# Autodesk Inventor assembly: Sun_StarwarsTrain
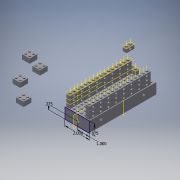
[picture p0: Inventor's stored thumbnail of the model, 180x180]
Saved by Autodesk Inventor 2016 (Build 200138000, 138)
## iProperties
Created: 2018-02-15
Part Number: Sun_StarwarsTrain
Document SubType Name: Assembly
Designer: sun01147
Author: sun01147
## Documents named in this file (6)
- E:\IED7_SunT\BrickTrainParts\Sun_StarwarsTrain.iam
- E:\IED7_SunT\BrickTrainParts\Caufield_Engine_Body_LEGO.ipt
- E:\IED7_SunT\BrickTrainParts\Sun_Bricks.ipt
- E:\IED7_SunT\BrickTrainParts\Yee_2x2Brick.ipt
- E:\IED7_SunT\BrickTrainParts\Sun_Bricks_MIR.ipt
- E:\IED7_SunT\BrickTrainParts\Sun_Bricks_MIR1.ipt
## Components (56 placed, 5 different names)
1. Caufield_Engine_Body_LEGO:1 — Mate:7, Mate:8, Mate:55
2. Sun_Bricks:1 — Mate:9, Flush:1, Mate:10, Flush:2, Flush:11
3. Sun_Bricks:2 — Mate:7, Mate:8, Mate:9, Flush:1, Mate:16
4. Sun_Bricks:3 — Mate:10, Flush:2, Flush:3, Mate:11, Mate:19
5. Sun_Bricks:4 — Flush:3, Mate:11, Mate:12, Flush:4, Mate:36
6. Yee_2x2Brick:1
7. Yee_2x2Brick:2
8. Yee_2x2Brick:3
9. Yee_2x2Brick:4
10. Sun_Bricks:5 — Mate:13, Flush:5, Mate:14, Flush:6
11. Sun_Bricks:6 — Mate:12, Flush:4, Mate:13, Flush:5
12. Sun_Bricks:7 — Mate:14, Flush:6, Mate:15, Flush:7
13. Sun_Bricks:8 — Mate:15, Flush:7, Flush:8, Flush:9, Flush:10, Mate:54, Flush:36
14. Sun_Bricks:9 — Mate:39, Mate:40, Mate:41
15. Sun_Bricks:10 — Flush:8, Flush:9, Flush:10
16. Sun_Bricks:11 — Mate:54, Mate:55, Flush:36
17. Sun_Bricks:12 — Mate:18, Flush:12
18. Sun_Bricks:13 — Mate:19, Flush:12, Flush:29
19. Sun_Bricks:14 — Mate:37, Mate:38
20. Sun_Bricks:15 — Mate:17, Flush:11, Mate:18
21. Sun_Bricks:16 — Mate:16, Mate:17
22. Sun_Bricks_MIR:1 — Flush:13, Mate:20, Flush:14, Mate:21, Flush:21
23. Sun_Bricks_MIR:2 — Flush:13, Mate:20, Mate:30
24. Sun_Bricks_MIR:3 — Flush:14, Mate:21, Mate:22, Flush:15, Mate:27
25. Sun_Bricks_MIR:4 — Mate:22, Flush:15, Flush:17, Mate:24, Mate:33
26. Sun_Bricks_MIR:5 — Flush:16, Mate:23, Flush:18, Mate:25
27. Sun_Bricks_MIR:6 — Flush:16, Mate:23, Flush:17, Mate:24
28. Sun_Bricks_MIR:7 — Flush:18, Mate:25, Flush:19, Mate:26
29. Sun_Bricks_MIR:8 — Flush:19, Mate:26
30. Sun_Bricks_MIR:9 — Flush:20, Mate:28
31. Sun_Bricks_MIR:10 — Flush:20, Mate:27, Flush:23
32. Sun_Bricks_MIR:11 — Mate:28, Flush:21, Mate:29
33. Sun_Bricks_MIR:12 — Mate:29, Mate:30
34. Sun_Bricks_MIR:13 — Flush:25
35. Sun_Bricks_MIR:14
36. Sun_Bricks_MIR:15 — Flush:24, Flush:25
37. Sun_Bricks_MIR:16 — Mate:33, Flush:23, Flush:24
38. Sun_Bricks_MIR:17 — Mate:39, Mate:40
39. Sun_Bricks_MIR:18 — Mate:37, Mate:38
40. Sun_Bricks_MIR:19 — Mate:42, Mate:45
41. Sun_Bricks_MIR:20 — Mate:36, Flush:29, Mate:43
42. Sun_Bricks:17 — Mate:43, Mate:44, Mate:45
43. Sun_Bricks:18 — Mate:41, Mate:42
44. Sun_Bricks:19 — Mate:46, Flush:30, Mate:47, Flush:31
45. Sun_Bricks:20 — Mate:47, Flush:31, Mate:48, Flush:32
46. Sun_Bricks:21 — Mate:48, Flush:32
47. Sun_Bricks:22
48. Sun_Bricks:23 — Mate:44, Mate:46, Flush:30
49. Sun_Bricks_MIR1:1 — Mate:49
50. Sun_Bricks_MIR1:2
51. Sun_Bricks_MIR1:3 — Mate:53
52. Sun_Bricks_MIR1:4 — Mate:49
53. Sun_Bricks_MIR1:5 — Flush:33, Mate:50, Flush:35, Mate:52
54. Sun_Bricks_MIR1:6 — Flush:33, Mate:50, Flush:34, Mate:51
55. Sun_Bricks_MIR1:7 — Flush:34, Mate:51
56. Sun_Bricks_MIR1:8 — Flush:35, Mate:52, Mate:53
## Relationships (85: Mate 49, Flush 36)
- Mate:7: Caufield_Engine_Body_LEGO:1 ↔ Sun_Bricks:2
- Mate:8: Caufield_Engine_Body_LEGO:1 ↔ Sun_Bricks:2
- Mate:9: Sun_Bricks:1 ↔ Sun_Bricks:2
- Flush:1: Sun_Bricks:1 ↔ Sun_Bricks:2
- Mate:10: Sun_Bricks:1 ↔ Sun_Bricks:3
- Flush:2: Sun_Bricks:1 ↔ Sun_Bricks:3
- Flush:3: Sun_Bricks:3 ↔ Sun_Bricks:4
- Mate:11: Sun_Bricks:3 ↔ Sun_Bricks:4
- Mate:12: Sun_Bricks:4 ↔ Sun_Bricks:6
- Flush:4: Sun_Bricks:4 ↔ Sun_Bricks:6
- Mate:13: Sun_Bricks:5 ↔ Sun_Bricks:6
- Flush:5: Sun_Bricks:5 ↔ Sun_Bricks:6
- Mate:14: Sun_Bricks:5 ↔ Sun_Bricks:7
- Flush:6: Sun_Bricks:5 ↔ Sun_Bricks:7
- Mate:15: Sun_Bricks:7 ↔ Sun_Bricks:8
- Flush:7: Sun_Bricks:7 ↔ Sun_Bricks:8
- Flush:8: Sun_Bricks:8 ↔ Sun_Bricks:10
- Flush:9: Sun_Bricks:8 ↔ Sun_Bricks:10
- Flush:10: Sun_Bricks:8 ↔ Sun_Bricks:10
- Mate:16: Sun_Bricks:2 ↔ Sun_Bricks:16
- Mate:17: Sun_Bricks:15 ↔ Sun_Bricks:16
- Flush:11: Sun_Bricks:1 ↔ Sun_Bricks:15
- Mate:18: Sun_Bricks:12 ↔ Sun_Bricks:15
- Mate:19: Sun_Bricks:3 ↔ Sun_Bricks:13
- Flush:12: Sun_Bricks:12 ↔ Sun_Bricks:13
- Flush:13: Sun_Bricks_MIR:1 ↔ Sun_Bricks_MIR:2
- Mate:20: Sun_Bricks_MIR:1 ↔ Sun_Bricks_MIR:2
- Flush:14: Sun_Bricks_MIR:1 ↔ Sun_Bricks_MIR:3
- Mate:21: Sun_Bricks_MIR:1 ↔ Sun_Bricks_MIR:3
- Mate:22: Sun_Bricks_MIR:3 ↔ Sun_Bricks_MIR:4
- Flush:15: Sun_Bricks_MIR:3 ↔ Sun_Bricks_MIR:4
- Flush:16: Sun_Bricks_MIR:5 ↔ Sun_Bricks_MIR:6
- Mate:23: Sun_Bricks_MIR:5 ↔ Sun_Bricks_MIR:6
- Flush:17: Sun_Bricks_MIR:4 ↔ Sun_Bricks_MIR:6
- Mate:24: Sun_Bricks_MIR:4 ↔ Sun_Bricks_MIR:6
- Flush:18: Sun_Bricks_MIR:5 ↔ Sun_Bricks_MIR:7
- Mate:25: Sun_Bricks_MIR:5 ↔ Sun_Bricks_MIR:7
- Flush:19: Sun_Bricks_MIR:7 ↔ Sun_Bricks_MIR:8
- Mate:26: Sun_Bricks_MIR:7 ↔ Sun_Bricks_MIR:8
- Flush:20: Sun_Bricks_MIR:9 ↔ Sun_Bricks_MIR:10
- Mate:27: Sun_Bricks_MIR:3 ↔ Sun_Bricks_MIR:10
- Mate:28: Sun_Bricks_MIR:9 ↔ Sun_Bricks_MIR:11
- Flush:21: Sun_Bricks_MIR:1 ↔ Sun_Bricks_MIR:11
- Mate:29: Sun_Bricks_MIR:11 ↔ Sun_Bricks_MIR:12
- Mate:30: Sun_Bricks_MIR:2 ↔ Sun_Bricks_MIR:12
- [Flush]: Sun_Bricks_MIR:13 ↔ Sun_Bricks_MIR:14
- [Mate]: Sun_Bricks_MIR:13 ↔ Sun_Bricks_MIR:15
- [Mate]: Sun_Bricks_MIR:15 ↔ Sun_Bricks_MIR:16
- Mate:33: Sun_Bricks_MIR:4 ↔ Sun_Bricks_MIR:16
- Flush:23: Sun_Bricks_MIR:10 ↔ Sun_Bricks_MIR:16
- Flush:24: Sun_Bricks_MIR:15 ↔ Sun_Bricks_MIR:16
- Flush:25: Sun_Bricks_MIR:13 ↔ Sun_Bricks_MIR:15
- [Flush]: Sun_Bricks_MIR:17 ↔ Sun_Bricks_MIR:18
- [Mate]: Sun_Bricks_MIR:17 ↔ Sun_Bricks_MIR:19
- [Mate]: Sun_Bricks_MIR:19 ↔ Sun_Bricks_MIR:20
- [Flush]: Sun_Bricks_MIR:19 ↔ Sun_Bricks_MIR:20
- [Flush]: Sun_Bricks_MIR:17 ↔ Sun_Bricks_MIR:19
- Mate:36: Sun_Bricks:4 ↔ Sun_Bricks_MIR:20
- Flush:29: Sun_Bricks:13 ↔ Sun_Bricks_MIR:20
- Mate:37: Sun_Bricks:14 ↔ Sun_Bricks_MIR:18
- Mate:38: Sun_Bricks:14 ↔ Sun_Bricks_MIR:18
- Mate:39: Sun_Bricks:9 ↔ Sun_Bricks_MIR:17
- Mate:40: Sun_Bricks:9 ↔ Sun_Bricks_MIR:17
- Mate:41: Sun_Bricks:9 ↔ Sun_Bricks:18
- Mate:42: Sun_Bricks_MIR:19 ↔ Sun_Bricks:18
- Mate:43: Sun_Bricks_MIR:20 ↔ Sun_Bricks:17
- Mate:44: Sun_Bricks:17 ↔ Sun_Bricks:23
- Mate:45: Sun_Bricks_MIR:19 ↔ Sun_Bricks:17
- Mate:46: Sun_Bricks:19 ↔ Sun_Bricks:23
- Flush:30: Sun_Bricks:19 ↔ Sun_Bricks:23
- Mate:47: Sun_Bricks:19 ↔ Sun_Bricks:20
- Flush:31: Sun_Bricks:19 ↔ Sun_Bricks:20
- Mate:48: Sun_Bricks:20 ↔ Sun_Bricks:21
- Flush:32: Sun_Bricks:20 ↔ Sun_Bricks:21
- Mate:49: Sun_Bricks_MIR1:1 ↔ Sun_Bricks_MIR1:4
- Flush:33: Sun_Bricks_MIR1:5 ↔ Sun_Bricks_MIR1:6
- Mate:50: Sun_Bricks_MIR1:5 ↔ Sun_Bricks_MIR1:6
- Flush:34: Sun_Bricks_MIR1:6 ↔ Sun_Bricks_MIR1:7
- Mate:51: Sun_Bricks_MIR1:6 ↔ Sun_Bricks_MIR1:7
- Flush:35: Sun_Bricks_MIR1:5 ↔ Sun_Bricks_MIR1:8
- Mate:52: Sun_Bricks_MIR1:5 ↔ Sun_Bricks_MIR1:8
- Mate:53: Sun_Bricks_MIR1:3 ↔ Sun_Bricks_MIR1:8
- Mate:54: Sun_Bricks:8 ↔ Sun_Bricks:11
- Mate:55: Caufield_Engine_Body_LEGO:1 ↔ Sun_Bricks:11
- Flush:36: Sun_Bricks:8 ↔ Sun_Bricks:11
## Named parameters: d54_d48 = 0 mm, d55_d50 = 0 mm, d56_d52 = 0 mm, d61_d54_d48 = 0 mm, d62_d55_d50 = 0 mm, d63_d56_d52 = 0 mm, d64_d59 = 0 mm, d65_d60 = 0 mm
